# Autodesk Inventor assembly: Cylinder Body Sub_Assy
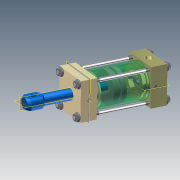
[picture p0: Inventor's stored thumbnail of the model, 180x180]
Saved by Autodesk Inventor 2011 (Build 150229000, 229)
## iProperties
Created: 2008-07-05
Part Number: Cylinder Body Sub_Assy
Document SubType Name: Assembly
Designer: normanpa
Mass: 1245.04 g
Surface Area: 688.692 cm^2
Volume: 165.976 cm^3
Density: 7.50134 g/cm^3
Author: normanpa
## Documents named in this file (10)
- C:\Program Files\Autodesk\Inventor 2011\Tutorial Files\Cylinder Clamp\Cylinder Body Sub_Assy.iam
- C:\Program Files\Autodesk\Inventor 2011\Tutorial Files\Cylinder Clamp\Cylinder Head Cover_Front.ipt
- C:\Program Files\Autodesk\Inventor 2011\Tutorial Files\Cylinder Clamp\Cylinder Body.ipt
- C:\Program Files\Autodesk\Inventor 2011\Tutorial Files\Cylinder Clamp\Cylinder Head Cover_Back.ipt
- C:\Program Files\Autodesk\Inventor 2011\Tutorial Files\Cylinder Clamp\M5 Threaded Rod.ipt
- C:\Program Files\Autodesk\Inventor 2011\Tutorial Files\Cylinder Clamp\ANSI B18.2.4.4M - M5 x 0.8.ipt
- C:\Program Files\Autodesk\Inventor 2011\Tutorial Files\Cylinder Clamp\Piston Rod.ipt
- C:\Program Files\Autodesk\Inventor 2011\Tutorial Files\Cylinder Clamp\Piston.ipt
- C:\Program Files\Autodesk\Inventor 2011\Tutorial Files\Cylinder Clamp\AS 1969 - M8(1).ipt
- C:\Program Files\Autodesk\Inventor 2011\Tutorial Files\Cylinder Clamp\ANSI B18.2.4.2M - M8x1.25 - 13.ipt
## Components (19 placed, 9 different names)
1. Cylinder Head Cover_Front:1 — Insert:1, Flush:1, Mate:1, Flush:2, Insert:3, Mate:2
2. Cylinder Body:1 — Insert:1, Insert:2
3. Cylinder Head Cover_Back:1 — Insert:2, Flush:1, Insert:4
4. Piston Rod:1 — Insert:5, Mate:2
5. Piston:1 — Insert:5, Insert:6
6. AS 1969 (External Tooth Lock Washer Type A) M8:1 — Insert:6, Insert:7
7. ANSI B18.2.4.2M M8x1.25:1 — Insert:7
8. M5 Threaded Rod:1 — Mate:1, Flush:2
9. Metric Hex Flange Nuts - Metric M5 x 0.8:1 — Insert:3
10. Metric Hex Flange Nuts - Metric M5 x 0.8:2 — Insert:4
11. M5 Threaded Rod:2
12. Metric Hex Flange Nuts - Metric M5 x 0.8:3
13. Metric Hex Flange Nuts - Metric M5 x 0.8:4
14. M5 Threaded Rod:3
15. Metric Hex Flange Nuts - Metric M5 x 0.8:5
16. Metric Hex Flange Nuts - Metric M5 x 0.8:6
17. M5 Threaded Rod:4
18. Metric Hex Flange Nuts - Metric M5 x 0.8:7
19. Metric Hex Flange Nuts - Metric M5 x 0.8:8
## Component patterns: (4 elements, first: M5 Threaded Rod:1 + Metric Hex Flange Nuts - Metric M5 x 0.8:1 + Metric Hex Flange Nuts - Metric M5 x 0.8:2)
## Relationships (11: Insert 7, Flush 2, Mate 2)
- Insert:1: Cylinder Head Cover_Front:1 ↔ Cylinder Body:1
- Insert:2: Cylinder Body:1 ↔ Cylinder Head Cover_Back:1
- Flush:1: Cylinder Head Cover_Front:1 ↔ Cylinder Head Cover_Back:1
- Mate:1: Cylinder Head Cover_Front:1 ↔ M5 Threaded Rod:1
- Flush:2 (5.5 mm): Cylinder Head Cover_Front:1 ↔ M5 Threaded Rod:1
- Insert:3: Cylinder Head Cover_Front:1 ↔ Metric Hex Flange Nuts - Metric M5 x 0.8:1
- Insert:4: Cylinder Head Cover_Back:1 ↔ Metric Hex Flange Nuts - Metric M5 x 0.8:2
- Insert:5: Piston Rod:1 ↔ Piston:1
- Insert:6: Piston:1 ↔ AS 1969 (External Tooth Lock Washer Type A) M8:1
- Insert:7: AS 1969 (External Tooth Lock Washer Type A) M8:1 ↔ ANSI B18.2.4.2M M8x1.25:1
- Mate:2: Cylinder Head Cover_Front:1 ↔ Piston Rod:1
